# Autodesk Inventor assembly: The Final Assembly
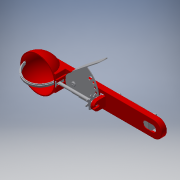
[picture p0: Inventor's stored thumbnail of the model, 180x180]
Saved by Autodesk Inventor 2016 (Build 200138000, 138)
## iProperties
Created: 2016-11-10
Part Number: The Final Assembly
Document SubType Name: Assembly
Designer: Muhammad
Author: Muhammad
## Documents named in this file (5)
- C:\Users\Muhammad\Desktop\Icecream scoop\The Final Assembly.iam
- C:\Users\Muhammad\Desktop\Icecream scoop\Ice Cream Assembly.iam
- C:\Users\Muhammad\Desktop\Icecream scoop\Battery holder.ipt
- C:\Users\Muhammad\Desktop\Icecream scoop\Battery.ipt
- C:\Users\Muhammad\Desktop\Icecream scoop\Metal icecream cutter redesign.ipt
## Components (4 placed, 4 different names)
1. Ice Cream Assembly:1 [sub-assembly] — Rigid:1, Mate:1
2. Battery holder:1 — Rigid:1, Insert:1
3. Battery:1 — Insert:1
4. Metal icecream cutter redesign:1 — Mate:1
## Relationships (3: WeldJoint 1, Insert 1, Mate 1)
- Rigid:1 [WeldJoint]: Ice Cream Assembly:1 ↔ Battery holder:1
- Insert:1: Battery holder:1 ↔ Battery:1
- Mate:1: Ice Cream Assembly:1 ↔ Metal icecream cutter redesign:1
